# Autodesk Inventor assembly: Vise
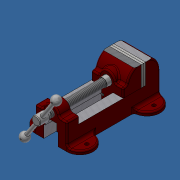
[picture p0: Inventor's stored thumbnail of the model, 180x180]
Saved by Autodesk Inventor 2022.4 (Build 264492010, 492A)
## iProperties
Created: 2006-01-18
Part Number: Vise
Document SubType Name: Assembly
Designer: PMiller
Mass: 5620.54 g
Surface Area: 1467.47 cm^2
Volume: 715.992 cm^3
Density: 7.85 g/cm^3
CN_MASS: 5.07
Author: PMiller
## iProperties of the stored document MemberDocs/xKlqmhksmKsey1xx4DpphmnrqCf
Created: 2006-01-18
Part Number: Vise
Document SubType Name: Assembly
Designer: PMiller
Mass: 5070.79 g
Surface Area: 1344.53 cm^2
Volume: 645.961 cm^3
Density: 7.85 g/cm^3
CN_MASS: 5.07
Author: PMiller
## iProperties of the stored document MemberDocs/xOqnar5ovPkk4bplyKeatyz31Kb
Created: 2006-01-18
Part Number: Vise
Document SubType Name: Assembly
Designer: PMiller
Mass: 5620.54 g
Surface Area: 1467.47 cm^2
Volume: 715.992 cm^3
Density: 7.85 g/cm^3
CN_MASS: 5.07
Author: PMiller
## Documents named in this file (10)
- U:\Inventor 2022 Training\_Designer Training\Inventor 2022 - Advanced Assembly\Practice Files\Model States\Vise_Model_States.iam
- U:\Inventor 2022 Training\_Designer Training\Inventor 2022 - Advanced Assembly\Practice Files\Model States\Base_Model_States.ipt
- U:\Inventor 2022 Training\_Designer Training\Inventor 2022 - Advanced Assembly\Practice Files\Model States\Sliding_Jaw.ipt
- U:\Inventor 2022 Training\_Designer Training\Inventor 2022 - Advanced Assembly\Practice Files\Model States\Screw_Sub_Model_States.iam
- U:\Inventor 2022 Training\_Designer Training\Inventor 2022 - Advanced Assembly\Practice Files\Model States\Collar.ipt
- U:\Inventor 2022 Training\_Designer Training\Inventor 2022 - Advanced Assembly\Practice Files\Model States\Jaw_Plate.ipt
- U:\Inventor 2022 Training\_Designer Training\Inventor 2022 - Advanced Assembly\Practice Files\Model States\Set_Screw.ipt
- U:\Inventor 2022 Training\_Designer Training\Inventor 2022 - Advanced Assembly\Practice Files\Model States\Slide_Key.ipt
- U:\Inventor 2022 Training\_Designer Training\Inventor 2022 - Advanced Assembly\Practice Files\Model States\Special_Key.ipt
- U:\Inventor 2022 Training\_Designer Training\Inventor 2022 - Advanced Assembly\Practice Files\Model States\1_4-0.75-UNC.ipt
## Components (15 placed, 9 different names)
1. Base_Model_States:1 — Flush:1, Flush:2, Insert:1, Insert:2, Mate:2, Mate:4
2. Sliding_Jaw:1 — Flush:1, Flush:2, Insert:3, Insert:4, Insert:11, Mate:1, Mate:3, Mate:5, Mate:6, Insert:12, Insert:13
3. Screw_Sub_Model_States:1 [sub-assembly] — Insert:9, Insert:10
4. Collar:1 — Insert:10, Insert:11
5. Jaw_Plate:1 — Insert:3, Insert:4, Insert:7, Insert:8, Mate:7
6. Jaw_Plate:2 — Insert:1, Insert:2, Insert:5, Insert:6, Mate:7
7. Set_Screw:1 — Insert:12
8. Set_Screw:2 — Insert:13
9. Slide_Key:1 — Mate:1, Mate:2, Mate:6
10. Slide_Key:2 — Mate:3, Mate:4, Mate:5
11. Special_Key:1 — Insert:9
12. Cross Recessed Flat Countersunk Head Machine Screw - Type I - Inch 1/4-20 x 3/4:1 — Insert:7
13. Cross Recessed Flat Countersunk Head Machine Screw - Type I - Inch 1/4-20 x 3/4:2 — Insert:8
14. Cross Recessed Flat Countersunk Head Machine Screw - Type I - Inch 1/4-20 x 3/4:3 — Insert:5
15. Cross Recessed Flat Countersunk Head Machine Screw - Type I - Inch 1/4-20 x 3/4:4 — Insert:6
## Relationships (22: Insert 13, Mate 7, Flush 2)
- Flush:1: Base_Model_States:1 ↔ Sliding_Jaw:1
- Flush:2: Base_Model_States:1 ↔ Sliding_Jaw:1
- Insert:1: Base_Model_States:1 ↔ Jaw_Plate:2
- Insert:2: Base_Model_States:1 ↔ Jaw_Plate:2
- Insert:3: Sliding_Jaw:1 ↔ Jaw_Plate:1
- Insert:4: Sliding_Jaw:1 ↔ Jaw_Plate:1
- Insert:5: Jaw_Plate:2 ↔ Cross Recessed Flat Countersunk Head Machine Screw - Type I - Inch 1/4-20 x 3/4:3
- Insert:6: Jaw_Plate:2 ↔ Cross Recessed Flat Countersunk Head Machine Screw - Type I - Inch 1/4-20 x 3/4:4
- Insert:7: Jaw_Plate:1 ↔ Cross Recessed Flat Countersunk Head Machine Screw - Type I - Inch 1/4-20 x 3/4:1
- Insert:8: Jaw_Plate:1 ↔ Cross Recessed Flat Countersunk Head Machine Screw - Type I - Inch 1/4-20 x 3/4:2
- Insert:9: Screw_Sub_Model_States:1 ↔ Special_Key:1
- Insert:10: Screw_Sub_Model_States:1 ↔ Collar:1
- Insert:11 (-11.1125 mm): Sliding_Jaw:1 ↔ Collar:1
- Mate:1: Sliding_Jaw:1 ↔ Slide_Key:1
- Mate:2: Base_Model_States:1 ↔ Slide_Key:1
- Mate:3: Sliding_Jaw:1 ↔ Slide_Key:2
- Mate:4: Base_Model_States:1 ↔ Slide_Key:2
- Mate:5: Sliding_Jaw:1 ↔ Slide_Key:2
- Mate:6: Sliding_Jaw:1 ↔ Slide_Key:1
- Insert:12: Sliding_Jaw:1 ↔ Set_Screw:1
- Insert:13: Sliding_Jaw:1 ↔ Set_Screw:2
- Mate:7: Jaw_Plate:1 ↔ Jaw_Plate:2
